# Autodesk Inventor assembly: rotula
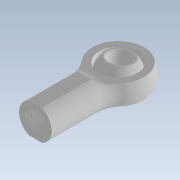
[picture p0: Inventor's stored thumbnail of the model, 180x180]
Saved by Autodesk Inventor 2021 (Build 250183000, 183)
## iProperties
Created: 2021-07-07
Part Number: rotula
Document SubType Name: Assembly
Designer: Andrés Holguín
Author: Andrés Holguín
## Documents named in this file (3)
- C:\Users\andre\Documents\GitHub\Dis.-Mecatronico-E6\inventor proyecto\Motores y reductores\rotula.iam
- C:\Users\andre\Documents\GitHub\Dis.-Mecatronico-E6\inventor proyecto\Motores y reductores\Rotula60645K731_STEEL BALL JOINT ROD END.ipt
- C:\Users\andre\Documents\GitHub\Dis.-Mecatronico-E6\inventor proyecto\Motores y reductores\Rotula60645K731_STEEL BALL JOINT ROD END_1.ipt
## Components (2 placed, 2 different names)
1. Rotula60645K731_STEEL BALL JOINT ROD END:1 — Ball:1
2. Rotula60645K731_STEEL BALL JOINT ROD END_1:1 — Ball:1
## Relationships (1: BallJoint 1)
- Ball:1: Rotula60645K731_STEEL BALL JOINT ROD END:1 ↔ Rotula60645K731_STEEL BALL JOINT ROD END_1:1
